# Autodesk Inventor assembly: ArmAssembly
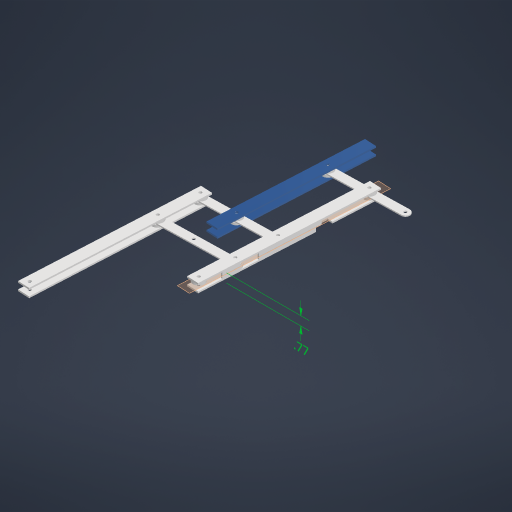
[picture p0: Inventor's stored thumbnail of the model, 512x512]
Saved by Autodesk Inventor 2024.2 (Build 282272000, 272)
## iProperties
Created: 2024-01-04
Part Number: ArmAssembly
Document SubType Name: Assembly
Designer: student
Author: student
## Documents named in this file (6)
- C:\Users\ctam0\Downloads\TRACER DOCUMENTS 1-13-2024\Arm Completed\ArmAssembly.iam
- C:\Users\ctam0\Downloads\TRACER DOCUMENTS 1-13-2024\Arm Completed\ArmPart1.ipt
- C:\Users\ctam0\Downloads\TRACER DOCUMENTS 1-13-2024\Arm Completed\ArmPart2.ipt
- C:\Users\ctam0\Downloads\TRACER DOCUMENTS 1-13-2024\Arm Completed\ArmPart3.ipt
- C:\Users\ctam0\Downloads\TRACER DOCUMENTS 1-13-2024\Arm Completed\ArmSpacer.ipt
- C:\Users\ctam0\Downloads\TRACER DOCUMENTS 1-13-2024\Arm Completed\ArmConnector1.ipt
## Components (19 placed, 5 different names)
1. ArmPart1:1 — Mate:9, Mate:10, Mate:13, Mate:19, Mate:66, Mate:68, Mate:69, Mate:72, Mate:73, Mate:78
2. ArmPart2:1 — Mate:64, Mate:65, Mate:67, Mate:71
3. ArmSpacer:1 — Mate:11, Mate:12, Mate:13
4. ArmSpacer:2 — Mate:9, Mate:10
5. ArmConnector1:2 — Mate:11, Mate:12, Mate:20, Mate:21, Mate:22, Mate:23, Mate:73
6. ArmSpacer:3 — Mate:16, Mate:17, Mate:19, Mate:72
7. ArmConnector1:3 — Mate:16, Mate:17, Mate:26, Mate:27, Mate:28, Mate:29, Mate:71, Mate:79, Mate:80, Mate:81, Mate:82
8. ArmSpacer:5 — Mate:28, Mate:29, Insert:3
9. ArmSpacer:6 — Mate:20, Mate:21, Insert:4
10. ArmSpacer:7 — Mate:81, Mate:82
11. ArmSpacer:8 — Mate:58, Mate:59
12. ArmSpacer:9 — Mate:22, Mate:23
13. ArmSpacer:10 — Mate:26, Mate:27
14. ArmSpacer:11 — Mate:56, Mate:57, Mate:64, Mate:65, Mate:67
15. ArmSpacer:12 — Mate:61, Mate:66, Mate:69, Mate:70, Mate:78
16. ArmSpacer:13 — Mate:79, Mate:80
17. ArmSpacer:14 — Mate:63, Mate:68
18. ArmConnector1:4 — Mate:56, Mate:57, Mate:58, Mate:59, Mate:61, Mate:63, Mate:70
19. ArmPart3:1 — Insert:3, Insert:4
## Relationships (39: Mate 37, Insert 2)
- Mate:9: ArmPart1:1 ↔ ArmSpacer:2
- Mate:10: ArmPart1:1 ↔ ArmSpacer:2
- Mate:11: ArmSpacer:1 ↔ ArmConnector1:2
- Mate:12: ArmSpacer:1 ↔ ArmConnector1:2
- Mate:13: ArmPart1:1 ↔ ArmSpacer:1
- Mate:16: ArmSpacer:3 ↔ ArmConnector1:3
- Mate:17: ArmSpacer:3 ↔ ArmConnector1:3
- Mate:19: ArmPart1:1 ↔ ArmSpacer:3
- Mate:20: ArmConnector1:2 ↔ ArmSpacer:6
- Mate:21: ArmConnector1:2 ↔ ArmSpacer:6
- Mate:22: ArmConnector1:2 ↔ ArmSpacer:9
- Mate:23: ArmConnector1:2 ↔ ArmSpacer:9
- Mate:26: ArmConnector1:3 ↔ ArmSpacer:10
- Mate:27: ArmConnector1:3 ↔ ArmSpacer:10
- Mate:28: ArmConnector1:3 ↔ ArmSpacer:5
- Mate:29: ArmConnector1:3 ↔ ArmSpacer:5
- Mate:56: ArmSpacer:11 ↔ ArmConnector1:4
- Mate:57: ArmSpacer:11 ↔ ArmConnector1:4
- Mate:58: ArmSpacer:8 ↔ ArmConnector1:4
- Mate:59: ArmSpacer:8 ↔ ArmConnector1:4
- Mate:61: ArmSpacer:12 ↔ ArmConnector1:4
- Mate:63: ArmSpacer:14 ↔ ArmConnector1:4
- Mate:64: ArmPart2:1 ↔ ArmSpacer:11
- Mate:65: ArmPart2:1 ↔ ArmSpacer:11
- Mate:66: ArmPart1:1 ↔ ArmSpacer:12
- Mate:67: ArmPart2:1 ↔ ArmSpacer:11
- Mate:68: ArmPart1:1 ↔ ArmSpacer:14
- Mate:69: ArmPart1:1 ↔ ArmSpacer:12
- Mate:70: ArmSpacer:12 ↔ ArmConnector1:4
- Insert:3: ArmSpacer:5 ↔ ArmPart3:1
- Insert:4: ArmSpacer:6 ↔ ArmPart3:1
- Mate:71: ArmPart2:1 ↔ ArmConnector1:3
- Mate:72: ArmPart1:1 ↔ ArmSpacer:3
- Mate:73: ArmPart1:1 ↔ ArmConnector1:2
- Mate:78: ArmPart1:1 ↔ ArmSpacer:12
- Mate:79: ArmConnector1:3 ↔ ArmSpacer:13
- Mate:80: ArmConnector1:3 ↔ ArmSpacer:13
- Mate:81: ArmConnector1:3 ↔ ArmSpacer:7
- Mate:82: ArmConnector1:3 ↔ ArmSpacer:7
